# Autodesk Inventor assembly: SimpleDesignV1 - 01
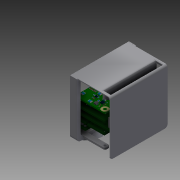
[picture p0: Inventor's stored thumbnail of the model, 180x180]
Saved by Autodesk Inventor 2015 (Build 190159000, 159)
## iProperties
Created: 2015-07-12
Part Number: SimpleDesignV1 - 01
Document SubType Name: Assembly
Designer: -
Author: -
## Documents named in this file (8)
- C:\Users\spichelh\Documents\GitHub\beta-hardware\Enclosure\SimpleDesign01\SimpleDesignV1 - 01.iam
- C:\Users\spichelh\Documents\GitHub\beta-hardware\Enclosure\Version 002\PCB Stack Concept V03 02.iam
- C:\Users\spichelh\Documents\GitHub\beta-hardware\Enclosure\SimpleDesign01\Mount-U-01.ipt
- C:\Users\spichelh\Documents\GitHub\beta-hardware\Enclosure\Version 002\Cooler.ipt
- C:\Users\spichelh\Documents\GitHub\beta-hardware\Enclosure\SimpleDesign01\SimpleFrontLeftPlate.ipt
- C:\Users\spichelh\Documents\GitHub\beta-hardware\Enclosure\SimpleDesign01\SimpleFrontRightPlate.ipt
- C:\Users\spichelh\Documents\GitHub\beta-hardware\Enclosure\SimpleDesign01\SimpleBackPlate.ipt
- C:\Users\spichelh\Documents\GitHub\beta-hardware\Enclosure\SimpleDesign01\E Mount.ipt
## Components (7 placed, 7 different names)
1. PCB Stack Concept V03 02:1 [sub-assembly] — Flush:1, Mate:1, Mate:2
2. Mount-U-01:1 — Flush:1, Mate:1, Mate:2, Mate:3, Flush:2, Flush:3, Flush:4, Flush:5, Flush:8, Flush:9, Flush:10, Flush:11, Mate:4, Flush:13, Mate:6
3. Cooler:1 — Mate:3
4. SimpleFrontLeftPlate:1 — Flush:2, Flush:3, Flush:9, Flush:10, Mate:5, Flush:14
5. SimpleFrontRightPlate:1 — Flush:4, Flush:5, Flush:8, Flush:11
6. SimpleBackPlate:1 — Mate:5, Flush:13, Flush:14
7. E Mount:1 — Mate:6
## Relationships (17: Flush 11, Mate 6)
- Flush:1: PCB Stack Concept V03 02:1 ↔ Mount-U-01:1
- Mate:1: PCB Stack Concept V03 02:1 ↔ Mount-U-01:1
- Mate:2 (1 mm): PCB Stack Concept V03 02:1 ↔ Mount-U-01:1
- Mate:3: Mount-U-01:1 ↔ Cooler:1
- Flush:2: Mount-U-01:1 ↔ SimpleFrontLeftPlate:1
- Flush:3: Mount-U-01:1 ↔ SimpleFrontLeftPlate:1
- Flush:4: Mount-U-01:1 ↔ SimpleFrontRightPlate:1
- Flush:5: Mount-U-01:1 ↔ SimpleFrontRightPlate:1
- Flush:8: Mount-U-01:1 ↔ SimpleFrontRightPlate:1
- Flush:9: Mount-U-01:1 ↔ SimpleFrontLeftPlate:1
- Flush:10: Mount-U-01:1 ↔ SimpleFrontLeftPlate:1
- Flush:11: Mount-U-01:1 ↔ SimpleFrontRightPlate:1
- Mate:4: Mount-U-01:1
- Mate:5: SimpleFrontLeftPlate:1 ↔ SimpleBackPlate:1
- Flush:13: Mount-U-01:1 ↔ SimpleBackPlate:1
- Flush:14: SimpleFrontLeftPlate:1 ↔ SimpleBackPlate:1
- Mate:6: Mount-U-01:1 ↔ E Mount:1
